# Autodesk Inventor assembly: Base
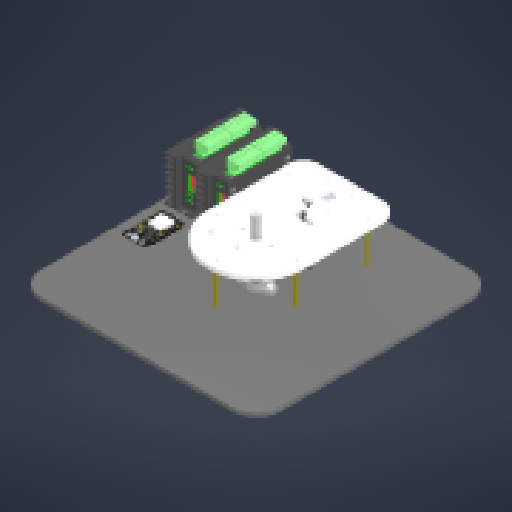
[picture p0: Inventor's stored thumbnail of the model, 512x512]
Saved by Autodesk Inventor 2023 (Build 270158000, 158)
## iProperties
Created: 2023-09-06
Part Number: Base
Document SubType Name: Assembly
Designer: philo
Sending System: Autodesk Inventor 2023
Preprocessor: ST-DEVELOPER v19
Title: C:\Users\philo\OneDrive\Desktop\HK1-2024\TT ROBOT\3DVer2\ROBOT_1_2.stp
Author: philo
## Documents named in this file (14)
- C:\Users\philo\OneDrive\Desktop\HK1-2024\TT ROBOT\02_3D_design_new\Base.iam
- C:\Users\philo\OneDrive\Desktop\HK1-2024\TT ROBOT\02_3D_design_new\DeRobot.ipt
- C:\Users\philo\OneDrive\Desktop\HK1-2024\TT ROBOT\02_3D_design_new\Detron.ipt
- C:\Users\philo\OneDrive\Desktop\HK1-2024\TT ROBOT\02_3D_design_new\goidoObi.ipt
- C:\Users\philo\OneDrive\Desktop\HK1-2024\TT ROBOT\02_3D_design_new\truday.ipt
- C:\Users\philo\OneDrive\Desktop\HK1-2024\TT ROBOT\02_3D_design_new\gt2_60teeth.iam
- C:\Users\philo\OneDrive\Desktop\HK1-2024\TT ROBOT\02_3D_design_new\M3 x 5mm.ipt
- C:\Users\philo\OneDrive\Desktop\HK1-2024\TT ROBOT\02_3D_design_new\Tb6600.ipt
- C:\Users\philo\OneDrive\Desktop\HK1-2024\TT ROBOT\02_3D_design_new\ESP-WROOM32.iam
- C:\Users\philo\OneDrive\Desktop\HK1-2024\TT ROBOT\02_3D_design_new\gt2smooth.ipt
- C:\Users\philo\OneDrive\Desktop\HK1-2024\TT ROBOT\02_3D_design_new\trudong5mm.ipt
- C:\Users\philo\OneDrive\Desktop\HK1-2024\TT ROBOT\02_3D_design_new\trucdogt2.ipt
- C:\Users\philo\OneDrive\Desktop\HK1-2024\TT ROBOT\02_3D_design_new\HALL.ipt
- C:\Users\philo\OneDrive\Desktop\HK1-2024\TT ROBOT\02_3D_design_new\namcham.ipt
## Components (22 placed, 13 different names)
1. DeRobot:1 — Mate:81, Mate:82, Mate:83, Mate:84, Mate:85, Mate:86, Mate:87, Mate:90, Mate:91, Mate:92, Mate:95, Flush:16, Mate:174, Mate:175
2. Detron:1 — Mate:81, Mate:94, Mate:95
3. goidoObi:1 — Mate:93, Mate:94
4. goidoObi:2 — Mate:89, Mate:92
5. truday:1 — Mate:87, Mate:88, Mate:93, Flush:16
6. gt2_60teeth:1 [sub-assembly] — Mate:88, Mate:89
7. M3 x 5mm:1
8. M3 x 5mm:6
9. M3 x 5mm:7 — Mate:90
10. M3 x 5mm:8 — Mate:91
11. Tb6600:1 — Mate:174
12. Tb6600:2 — Mate:175
13. ESP-WROOM32:1 [sub-assembly]
14. gt2smooth:1 — Mate:99
15. trudong5mm:4 — Mate:84
16. trudong5mm:5 — Mate:82
17. trudong5mm:6 — Mate:85
18. trudong5mm:8 — Mate:86
19. trudong5mm:9 — Mate:83
20. trucdogt2:1 — Mate:99
21. HALL:1
22. namcham:1
## Relationships (19: Mate 18, Flush 1)
- Mate:81 (45 mm): DeRobot:1 ↔ Detron:1
- Mate:82: DeRobot:1 ↔ trudong5mm:5
- Mate:83: DeRobot:1 ↔ trudong5mm:9
- Mate:84: DeRobot:1 ↔ trudong5mm:4
- Mate:85: DeRobot:1 ↔ trudong5mm:6
- Mate:86: DeRobot:1 ↔ trudong5mm:8
- Mate:87: DeRobot:1 ↔ truday:1
- Mate:88: truday:1 ↔ gt2_60teeth:1
- Mate:89: goidoObi:2 ↔ gt2_60teeth:1
- Mate:90: DeRobot:1 ↔ M3 x 5mm:7
- Mate:91: DeRobot:1 ↔ M3 x 5mm:8
- Mate:92: DeRobot:1 ↔ goidoObi:2
- Mate:93: goidoObi:1 ↔ truday:1
- Mate:94: Detron:1 ↔ goidoObi:1
- Mate:95: DeRobot:1 ↔ Detron:1
- Mate:99: gt2smooth:1 ↔ trucdogt2:1
- Flush:16: DeRobot:1 ↔ truday:1
- Mate:174: DeRobot:1 ↔ Tb6600:1
- Mate:175: DeRobot:1 ↔ Tb6600:2
